# Autodesk Inventor assembly: Assembly11
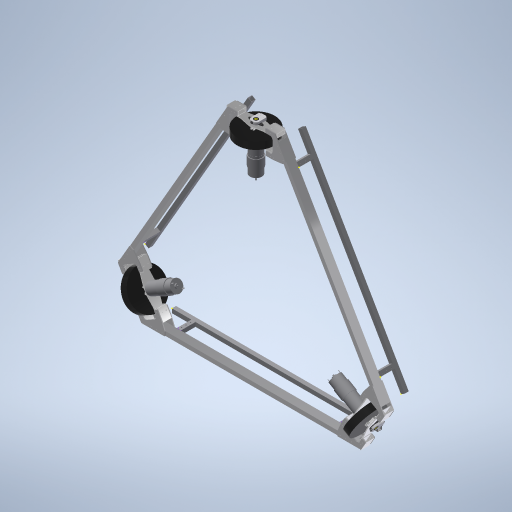
[picture p0: Inventor's stored thumbnail of the model, 512x512]
Saved by Autodesk Inventor 2023 (Build 270158000, 158)
## iProperties
Created: 2022-04-09
Part Number: Assembly11
Material: 一般
Document SubType Name: Assembly
Designer: yuta
Author: yuta
## Documents named in this file (4)
- C:\Users\yuta\Documents\NHK\Assembly11.iam
- C:\Users\yuta\Downloads\オムニホイール\オムニホイール\3輪オムニホイール.iam
- C:\Users\yuta\Documents\NHK\足2.ipt
- C:\Users\yuta\Documents\NHK\足3.ipt
## Components (10 placed, 3 different names)
1. 3輪オムニホイール:1 [sub-assembly] — メイト:1, フラッシュ:1, フラッシュ:2, メイト:2, フラッシュ:3, フラッシュ:4, メイト:3, フラッシュ:5, フラッシュ:6, メイト:4, フラッシュ:7, フラッシュ:8, メイト:5, フラッシュ:9, フラッシュ:10, メイト:6, フラッシュ:11, フラッシュ:12, フラッシュ:14, フラッシュ:16, フラッシュ:17, フラッシュ:18
2. 足2:1 — メイト:2, フラッシュ:3, フラッシュ:4, メイト:9
3. 足2:2 — メイト:1, フラッシュ:1, フラッシュ:2
4. 足2:3 — メイト:5, フラッシュ:9, フラッシュ:10, メイト:7
5. 足2:4 — メイト:6, フラッシュ:11, フラッシュ:12, フラッシュ:13
6. 足2:5 — メイト:4, フラッシュ:7, フラッシュ:8
7. 足2:6 — メイト:3, フラッシュ:5, フラッシュ:6, メイト:8, フラッシュ:15
8. 足3:1 — メイト:7, フラッシュ:13, フラッシュ:14
9. 足3:2 — メイト:9, フラッシュ:17, フラッシュ:18
10. 足3:3 — メイト:8, フラッシュ:15, フラッシュ:16
## Relationships (27: Flush 18, Mate 9)
- メイト:1 [Mate]: 3輪オムニホイール:1 ↔ 足2:2
- フラッシュ:1 [Flush]: 3輪オムニホイール:1 ↔ 足2:2
- フラッシュ:2 [Flush] (70 mm): 3輪オムニホイール:1 ↔ 足2:2
- メイト:2 [Mate]: 3輪オムニホイール:1 ↔ 足2:1
- フラッシュ:3 [Flush]: 3輪オムニホイール:1 ↔ 足2:1
- フラッシュ:4 [Flush] (70 mm): 3輪オムニホイール:1 ↔ 足2:1
- メイト:3 [Mate]: 3輪オムニホイール:1 ↔ 足2:6
- フラッシュ:5 [Flush]: 3輪オムニホイール:1 ↔ 足2:6
- フラッシュ:6 [Flush] (70 mm): 3輪オムニホイール:1 ↔ 足2:6
- メイト:4 [Mate]: 3輪オムニホイール:1 ↔ 足2:5
- フラッシュ:7 [Flush]: 3輪オムニホイール:1 ↔ 足2:5
- フラッシュ:8 [Flush] (70 mm): 3輪オムニホイール:1 ↔ 足2:5
- メイト:5 [Mate]: 3輪オムニホイール:1 ↔ 足2:3
- フラッシュ:9 [Flush]: 3輪オムニホイール:1 ↔ 足2:3
- フラッシュ:10 [Flush] (70 mm): 3輪オムニホイール:1 ↔ 足2:3
- メイト:6 [Mate]: 3輪オムニホイール:1 ↔ 足2:4
- フラッシュ:11 [Flush]: 3輪オムニホイール:1 ↔ 足2:4
- フラッシュ:12 [Flush] (70 mm): 3輪オムニホイール:1 ↔ 足2:4
- メイト:7 [Mate]: 足2:3 ↔ 足3:1
- フラッシュ:13 [Flush]: 足2:4 ↔ 足3:1
- フラッシュ:14 [Flush]: 3輪オムニホイール:1 ↔ 足3:1
- メイト:8 [Mate]: 足2:6 ↔ 足3:3
- フラッシュ:15 [Flush]: 足2:6 ↔ 足3:3
- フラッシュ:16 [Flush]: 3輪オムニホイール:1 ↔ 足3:3
- メイト:9 [Mate]: 足2:1 ↔ 足3:2
- フラッシュ:17 [Flush]: 3輪オムニホイール:1 ↔ 足3:2
- フラッシュ:18 [Flush]: 3輪オムニホイール:1 ↔ 足3:2
